# Autodesk Inventor assembly: Finger
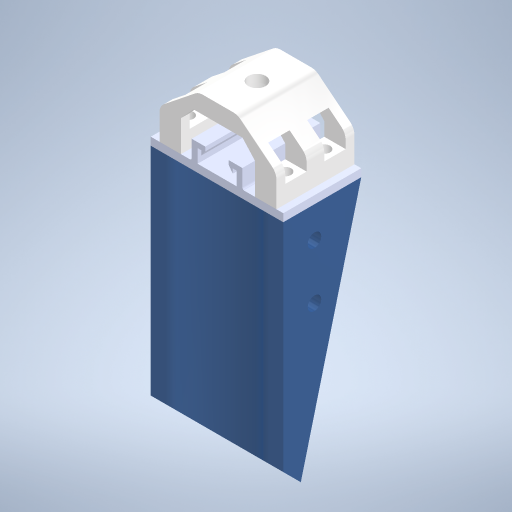
[picture p0: Inventor's stored thumbnail of the model, 512x512]
Saved by Autodesk Inventor 2024.2 (Build 282272000, 272)
## iProperties
Created: 2026-04-14
Part Number: Finger
Document SubType Name: Assembly
Designer: Admin
Author: 1.5:1
Title: Garra
Subject: 2
## Documents named in this file (4)
- C:\Users\Admin\Documents\GitHub\ManipuladorCartesiano\DiseñoMecánico\Assemblies\Finger.iam
- C:\Users\Admin\Documents\GitHub\ManipuladorCartesiano\DiseñoMecánico\AuxiliarPieces\ClawPrinted\GripperSupport.ipt
- C:\Users\Admin\Documents\GitHub\ManipuladorCartesiano\DiseñoMecánico\AuxiliarPieces\ClawPrinted\Gripper.ipt
- C:\Users\Admin\Documents\GitHub\ManipuladorCartesiano\DiseñoMecánico\AuxiliarPieces\ClawAlPieces\SliderPiece.ipt
## Components (3 placed, 3 different names)
1. GripperSupport:1 — Mate:4, Mate:5, Mate:6
2. Gripper:1 — Mate:1, Mate:2, Mate:3, Mate:5, Mate:6
3. SliderPiece:1 — Mate:1, Mate:2, Mate:3, Mate:4
## Relationships (6: Mate 6)
- Mate:1: Gripper:1 ↔ SliderPiece:1
- Mate:2: Gripper:1 ↔ SliderPiece:1
- Mate:3: Gripper:1 ↔ SliderPiece:1
- Mate:4: GripperSupport:1 ↔ SliderPiece:1
- Mate:5: GripperSupport:1 ↔ Gripper:1
- Mate:6: GripperSupport:1 ↔ Gripper:1
